# Autodesk Inventor assembly: CONCELEAD HINGE 170 DEG FULL OVERLAY DP45_9.5 HD1 EURSCR
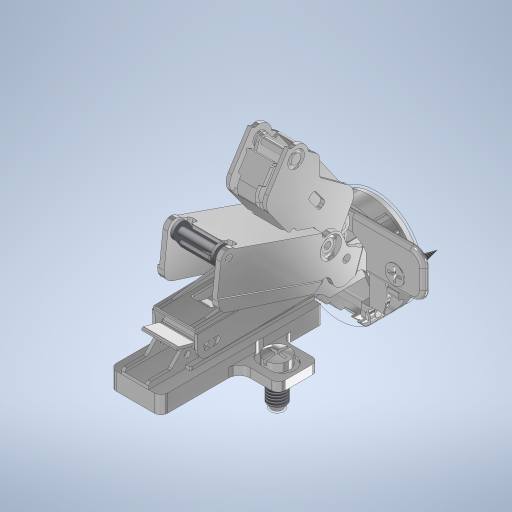
[picture p0: Inventor's stored thumbnail of the model, 512x512]
Saved by Autodesk Inventor 2024 (Build 280153000, 153)
## iProperties
Created: 2015-04-29
Part Number: CONCELEAD HINGE 170 DEG FULL OVERLAY DP45_9.5 HD1 EURSCR
Document SubType Name: Assembly
Designer: SauliusD
Author: SauliusD
## Documents named in this file (11)
- C:\W4INV 2024 Design\_LIBRARY\Hinges\CONCELEAD HINGE 170 DEG FULL OVERLAY\CONCELEAD HINGE 170 DEG FULL OVERLAY DP45_9.5 HD1 EURSCR.iam
- C:\W4INV 2024 Design\LIBRARY\Hinges\Parts\170 Deg Hinge Parts\Hinge 170 Degree Full Overlay.ipt
- C:\W4INV 2024 Design\LIBRARY\Hinges\Parts\170 Deg Hinge Parts\Lever 1 170 deg Hinge.ipt
- C:\W4INV 2024 Design\LIBRARY\Hinges\Parts\170 Deg Hinge Parts\Lever 2 170 deg Hinge.ipt
- C:\W4INV 2024 Design\LIBRARY\Hinges\Parts\170 Deg Hinge Parts\Lever 3 170 deg Hinge.ipt
- C:\W4INV 2024 Design\LIBRARY\Hinges\Parts\170 Deg Hinge Parts\Lever 4 170 deg Hinge.ipt
- C:\W4INV 2024 Design\LIBRARY\Hinges\CONCELEAD HINGE 170 DEG FULL OVERLAY.iam
- C:\W4INV 2024 Design\_LIBRARY\Hinges\Parts\170 Deg Hinge Parts\170 deg Hinge Cup\170 deg Hinge Cup DP45_9.5 HD1.ipt
- C:\W4INV 2024 Design\_LIBRARY\Hinges\Parts\Concelead Hinge\Duomatic mounting plate _\Duomatic mounting plate H6 FX EURSCR.ipt
- C:\W4INV 2023 Design\LIBRARY\Hinges\Parts\170 Deg Hinge Parts\170 deg Hinge Cup.ipt
- C:\W4INV 2023 Design\LIBRARY\Hinges\Parts\Concelead Hinge\Duomatic mounting plate .ipt
## Components (7 placed, 7 different names)
1. Hinge 170 Degree Full Overlay:1 — Mate:7, Mate:9, Mate:17, Mate:18, Mate:19
2. Lever 1 170 deg Hinge:1 — Mate:3, Mate:11, Mate:13
3. Lever 2 170 deg Hinge:1 — Mate:4, Mate:9, Mate:10, Mate:11
4. Lever 3 170 deg Hinge:1 — Mate:5, Mate:8, Mate:10, Mate:14
5. Lever 4 170 deg Hinge:1 — Mate:6, Mate:7, Mate:8
6. 170 deg Hinge Cup DP45_9.5 HD1:1 — Mate:12, Mate:13, Mate:14, Angle:1
7. Duomatic mounting plate H6 FX EURSCR:1 — Mate:15, Flush:2, Flush:3, Mate:18, Mate:19, Angle:1
## Relationships (19: Mate 16, Flush 2, Angle 1)
- Mate:3: Lever 1 170 deg Hinge:1
- Mate:4: Lever 2 170 deg Hinge:1
- Mate:5: Lever 3 170 deg Hinge:1
- Mate:6: Lever 4 170 deg Hinge:1
- Mate:7: Hinge 170 Degree Full Overlay:1 ↔ Lever 4 170 deg Hinge:1
- Mate:8: Lever 3 170 deg Hinge:1 ↔ Lever 4 170 deg Hinge:1
- Mate:9: Hinge 170 Degree Full Overlay:1 ↔ Lever 2 170 deg Hinge:1
- Mate:10: Lever 2 170 deg Hinge:1 ↔ Lever 3 170 deg Hinge:1
- Mate:11: Lever 1 170 deg Hinge:1 ↔ Lever 2 170 deg Hinge:1
- Mate:12: 170 deg Hinge Cup DP45_9.5 HD1:1
- Mate:13: Lever 1 170 deg Hinge:1 ↔ 170 deg Hinge Cup DP45_9.5 HD1:1
- Mate:14: Lever 3 170 deg Hinge:1 ↔ 170 deg Hinge Cup DP45_9.5 HD1:1
- Mate:15: Duomatic mounting plate H6 FX EURSCR:1
- Flush:2: Duomatic mounting plate H6 FX EURSCR:1
- Flush:3 (3.8 mm): Duomatic mounting plate H6 FX EURSCR:1
- Mate:17: Hinge 170 Degree Full Overlay:1
- Mate:18 (19.389 mm): Hinge 170 Degree Full Overlay:1 ↔ Duomatic mounting plate H6 FX EURSCR:1
- Mate:19 (10 mm): Hinge 170 Degree Full Overlay:1 ↔ Duomatic mounting plate H6 FX EURSCR:1
- Angle:1 (270 deg): 170 deg Hinge Cup DP45_9.5 HD1:1 ↔ Duomatic mounting plate H6 FX EURSCR:1
